# Autodesk Inventor assembly: Ensamble VirPong Prototipo Inicial
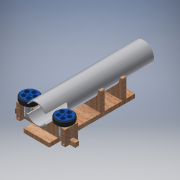
[picture p0: Inventor's stored thumbnail of the model, 180x180]
Saved by Autodesk Inventor 2016 SP2 (Build 200236200, 236)
## iProperties
Created: 2017-07-18
Part Number: Ensamble VirPong Prototipo Inicial
Material: Genérico
Document SubType Name: Assembly
Designer: ssant
Author: ssant
## Documents named in this file (8)
- C:\Users\ssant\Documents\My Works\Trabajos Varios\Proyectos\VirPong\CAD\Prototipo Inicial\Ensamble VirPong Prototipo Inicial.iam
- C:\Users\ssant\Documents\My Works\Trabajos Varios\Proyectos\VirPong\CAD\Prototipo Inicial\Base.ipt
- C:\Users\ssant\Documents\My Works\Trabajos Varios\Proyectos\VirPong\CAD\Prototipo Inicial\Soporte para Cañón.ipt
- C:\Users\ssant\Documents\My Works\Trabajos Varios\Proyectos\VirPong\CAD\Prototipo Inicial\Soporte para Motor 2.ipt
- C:\Users\ssant\Documents\My Works\Trabajos Varios\Proyectos\VirPong\CAD\Prototipo Inicial\Motor.ipt
- C:\Users\ssant\Documents\My Works\Trabajos Varios\Proyectos\VirPong\CAD\Prototipo Inicial\Tope para Motor.ipt
- C:\Users\ssant\Documents\My Works\Trabajos Varios\Proyectos\VirPong\CAD\Prototipo Inicial\Rueda.ipt
- C:\Users\ssant\Documents\My Works\Trabajos Varios\Proyectos\VirPong\CAD\Prototipo Inicial\Cañón.ipt
## Components (11 placed, 7 different names)
1. Base:1 — Coincidencia:1, Coincidencia:2, Nivelación:1, Nivelación:2, Coincidencia:3, Coincidencia:4, Coincidencia:6, Nivelación:3, Coincidencia:7, Nivelación:10
2. Soporte para Cañón:1 — Coincidencia:1, Nivelación:1, Coincidencia:3, Coincidencia:5, Coincidencia:8, Coincidencia:15
3. Soporte para Cañón:2 — Coincidencia:2, Nivelación:2, Coincidencia:4, Coincidencia:5, Coincidencia:17
4. Soporte para Motor 2:1 — Coincidencia:6, Nivelación:3, Coincidencia:7, Coincidencia:8, Coincidencia:11, Coincidencia:12, Nivelación:8, Coincidencia:13, Coincidencia:14, Nivelación:9, Coincidencia:16
5. Motor:1 — Coincidencia:10, Nivelación:6, Nivelación:7, Insertar:1
6. Motor:2 — Coincidencia:9, Nivelación:4, Nivelación:5, Insertar:2
7. Tope para Motor:1 — Coincidencia:10, Nivelación:6, Nivelación:7, Coincidencia:11, Coincidencia:12, Nivelación:8
8. Tope para Motor:2 — Coincidencia:9, Nivelación:4, Nivelación:5, Coincidencia:13, Coincidencia:14, Nivelación:9
9. Rueda:1 — Insertar:1
10. Rueda:2 — Insertar:2
11. Cañón:1 — Coincidencia:15, Coincidencia:16, Coincidencia:17, Nivelación:10
## Relationships (29: Mate 17, Flush 10, Insert 2)
- Coincidencia:1 [Mate]: Base:1 ↔ Soporte para Cañón:1
- Coincidencia:2 [Mate]: Base:1 ↔ Soporte para Cañón:2
- Nivelación:1 [Flush]: Base:1 ↔ Soporte para Cañón:1
- Nivelación:2 [Flush]: Base:1 ↔ Soporte para Cañón:2
- Coincidencia:3 [Mate]: Base:1 ↔ Soporte para Cañón:1
- Coincidencia:4 [Mate]: Base:1 ↔ Soporte para Cañón:2
- Coincidencia:5 [Mate]: Soporte para Cañón:1 ↔ Soporte para Cañón:2
- Coincidencia:6 [Mate]: Base:1 ↔ Soporte para Motor 2:1
- Nivelación:3 [Flush]: Base:1 ↔ Soporte para Motor 2:1
- Coincidencia:7 [Mate]: Base:1 ↔ Soporte para Motor 2:1
- Coincidencia:8 [Mate]: Soporte para Cañón:1 ↔ Soporte para Motor 2:1
- Coincidencia:9 [Mate]: Motor:2 ↔ Tope para Motor:2
- Nivelación:4 [Flush]: Motor:2 ↔ Tope para Motor:2
- Nivelación:5 [Flush] (-2.5 mm): Motor:2 ↔ Tope para Motor:2
- Coincidencia:10 [Mate]: Motor:1 ↔ Tope para Motor:1
- Nivelación:6 [Flush]: Motor:1 ↔ Tope para Motor:1
- Nivelación:7 [Flush] (-2.5 mm): Motor:1 ↔ Tope para Motor:1
- Coincidencia:11 [Mate]: Soporte para Motor 2:1 ↔ Tope para Motor:1
- Coincidencia:12 [Mate]: Soporte para Motor 2:1 ↔ Tope para Motor:1
- Nivelación:8 [Flush]: Soporte para Motor 2:1 ↔ Tope para Motor:1
- Coincidencia:13 [Mate]: Soporte para Motor 2:1 ↔ Tope para Motor:2
- Coincidencia:14 [Mate]: Soporte para Motor 2:1 ↔ Tope para Motor:2
- Nivelación:9 [Flush]: Soporte para Motor 2:1 ↔ Tope para Motor:2
- Insertar:1: Motor:1 ↔ Rueda:1
- Insertar:2: Motor:2 ↔ Rueda:2
- Coincidencia:15 [Mate]: Soporte para Cañón:1 ↔ Cañón:1
- Coincidencia:16 [Mate]: Soporte para Motor 2:1 ↔ Cañón:1
- Coincidencia:17 [Mate]: Soporte para Cañón:2 ↔ Cañón:1
- Nivelación:10 [Flush]: Base:1 ↔ Cañón:1
